(part 1 of 2)
# Autodesk Inventor assembly: Rebuild Chassis Assembly 26x28 Version with Shooter Tower
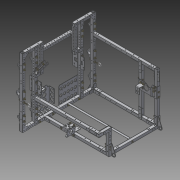
[picture p0: Inventor's stored thumbnail of the model, 180x180]
Saved by Autodesk Inventor 2014 SP1 (Build 180222100, 222)
## iProperties
Created: 2013-01-06
Part Number: Rebuild Chassis Assembly 26x28 Version with Shooter Tower
Document SubType Name: Assembly
Designer: Moses
Mass: 8941.51 g
Surface Area: 25286.9 cm^2
Volume: 3020.66 cm^3
Density: 2.96012 g/cm^3
Author: Moses
## Documents named in this file (57)
- C:\Users\Moses\Documents\Inventor\Sally Rebuild\Rebuild Sally\Rebuild Chassis Assembly 26x28 Version with Shooter Tower.iam
- C:\Users\Moses\Documents\Inventor\Sally Rebuild\Rebuild Sally\Chassis V1.500 Part3-mirror.ipt
- C:\Users\Moses\Documents\Inventor\Sally Rebuild\Rebuild Sally\Chassis V1.500 Part2.ipt
- C:\Users\Moses\Documents\Inventor\Sally Rebuild\Rebuild Sally\Chassis V1.500 Part3.ipt
- C:\Users\Moses\Documents\Inventor\Sally Rebuild\Rebuild Sally\Chassis Connector Plate V1.500.ipt
- C:\Users\Moses\Documents\Inventor\Sally Rebuild\Rebuild Sally\Chassis Corner Plate V1.500.ipt
- C:\Users\Moses\Documents\Inventor\Sally Rebuild\Rebuild Sally\Chassis Part4 (26x28).ipt
- C:\Users\Moses\Documents\Inventor\Sally Rebuild\Rebuild Sally\Chassis Part1 (26x28).ipt
- C:\Users\Moses\Documents\Inventor\Sally Rebuild\Rebuild Sally\Chassis Battery Mount Part1.ipt
- C:\Users\Moses\Documents\Inventor\Sally Rebuild\Rebuild Sally\Chassis Part9 (26x28).ipt
- C:\Users\Moses\Documents\Inventor\Sally Rebuild\Rebuild Sally\Chassis Part10 (26x28).ipt
- C:\Users\Moses\Documents\Inventor\Sally Rebuild\Rebuild Sally\Chassis Part 11 (26x28).ipt
- C:\Users\Moses\Documents\Inventor\Sally Rebuild\Rebuild Sally\Chassis Part 12 (26x28).ipt
- C:\Users\Moses\Documents\Inventor\Sally Rebuild\Rebuild Sally\Chassis Tower Bracket Part3.ipt
- C:\Users\Moses\Documents\Inventor\Sally Rebuild\Rebuild Sally\Chassis Tower Bracket Part2.ipt
- C:\Users\Moses\Documents\Inventor\Sally Rebuild\Rebuild Sally\Chassis Tower Bracket Part1.ipt
- C:\Users\Moses\Documents\Inventor\Sally Rebuild\Rebuild Sally\Rebuild Gusset 4.ipt
- C:\Users\Moses\Documents\Inventor\Sally Rebuild\Rebuild Sally\Rebuild Edge Mount 1.ipt
- C:\Users\Moses\Documents\Inventor\Sally Rebuild\Rebuild Sally\Rebuild Edge Mount 2.ipt
- C:\Users\Moses\Documents\Inventor\Sally Rebuild\Rebuild Sally\Rebuild Edge Mount 3.ipt
- C:\Users\Moses\Documents\Inventor\Sally Rebuild\Rebuild Sally\Rebuild Edge Mount 4.ipt
- C:\Users\Moses\Documents\Inventor\Sally Rebuild\Rebuild Sally\Rebuild Gusset.ipt
- C:\Users\Moses\Documents\Inventor\Sally Rebuild\Rebuild Sally\Rebuild Gusset 2.ipt
- C:\Users\Moses\Documents\Inventor\Sally Rebuild\Rebuild Sally\Gusset 3.ipt
- C:\Users\Moses\Documents\Inventor\Sally Rebuild\Rebuild Sally\Square Tube 6.ipt
- C:\Users\Moses\Documents\Inventor\Sally Rebuild\Rebuild Sally\Square Tube 3.ipt
- C:\Users\Moses\Documents\Inventor\Sally Rebuild\Rebuild Sally\Rebuild Shooter Tower Top Tube 2.ipt
- C:\Users\Moses\Documents\Inventor\Sally Rebuild\Rebuild Sally\Rebuild Gusset Connector 2.ipt
- C:\Users\Moses\Documents\Inventor\Sally Rebuild\Rebuild Sally\Rebuild Shooter Tower Top Tube 1.ipt
- C:\Users\Moses\Documents\Inventor\Sally Rebuild\Rebuild Sally\Rebuild Shooter Tower Motor Mount Tube.ipt
- C:\Users\Moses\Documents\Inventor\Sally Rebuild\Rebuild Sally\Shaft Mount V1.500 Drivetrain.ipt
- C:\Users\Moses\Documents\Inventor\Sally Rebuild\Rebuild Sally\Bearing Block V1.500 Drivetrain.ipt
- C:\Users\Moses\Documents\Inventor\Sally Rebuild\Rebuild Sally\Wheel Mount Support Plate - drive wheel.ipt
- C:\Users\Moses\Documents\Inventor\Sally Rebuild\Rebuild Sally\Wheel Mount Support Plate.ipt
- C:\Users\Moses\Documents\Inventor\Sally Rebuild\Rebuild Sally\Standard High-Strength Steel Cap Screw 0.25-20 Thread\Thread Length 0.75 - 1 in\2.000 in 91257A550\91257A550.ipt
- C:\Users\Moses\Documents\Inventor\Sally Rebuild\Rebuild Sally\Standard High-Strength Steel Cap Screw 0.25-20 Thread\90630A110.ipt
- C:\Users\Moses\Documents\Inventor\Sally Rebuild\Rebuild Sally\0.25x20 Washer.ipt
- C:\Users\Moses\Documents\Inventor\Sally Rebuild\Rebuild Sally\Standard High-Strength Steel Cap Screw 0.25-20 Thread\Thread Length 0.75 - 1 in\2.250 in 91257A551\91257A551.ipt
- C:\Users\Moses\Documents\Inventor\Sally Rebuild\Rebuild Sally\Standard High-Strength Steel Cap Screw 0.25-20 Thread\Thread Length 0.75 - 1 in\1.750 in 91257A548\91257A548.ipt
- C:\Users\Moses\Documents\Inventor\Sally Rebuild\Rebuild Sally\Rebuild Flange Bearing Mount Tower.ipt
- C:\Users\Moses\Documents\Inventor\Sally Rebuild\Rebuild Sally\Rebuild Flange Bearing Mount Tower Mirror.ipt
- C:\Users\Moses\Documents\Inventor\Sally Rebuild\Rebuild Sally\Mounting Bracket V1.500 - (toughbox-mini - sheet metal).ipt
- C:\Users\Moses\Documents\Inventor\Sally Rebuild\Rebuild Sally\Mounting Bracket V1.500 - (toughbox-mini - sheet metal - underside).ipt
- C:\Users\Moses\Documents\Inventor\Sally Rebuild\Rebuild Sally\Rebuild Mounting Board 3.ipt
- C:\Users\Moses\Documents\Inventor\Sally Rebuild\Rebuild Sally\Back Brace Mount V2.ipt
- C:\Users\Moses\Documents\Inventor\Sally Rebuild\Rebuild Sally\Circuit Breaker Mount.ipt
- C:\Users\Moses\Documents\Inventor\Sally Rebuild\Rebuild Sally\Standard High-Strength Steel Cap Screw 0.25-20 Thread\Fully Threaded\0.750 in 92620A540\92620A540.ipt
- C:\Users\Moses\Documents\Inventor\Sally Rebuild\Rebuild Sally\Rebuild Snowblower Motor Mount.ipt
- C:\Users\Moses\Documents\Inventor\Sally Rebuild\Rebuild Sally\Rebuild Encoder Mount 2.ipt
- C:\Users\Moses\Documents\Inventor\Sally Rebuild\Rebuild Sally\Standard High-Strength Steel Cap Screw 0.25-20 Thread\Fully Threaded\0.625 in 92620A539\92620A539.ipt
- C:\Users\Moses\Documents\Inventor\Sally Rebuild\Rebuild Sally\Chassis Back Electronics Protector Bar.ipt
- C:\Users\Moses\Documents\Inventor\Sally Rebuild\Rebuild Sally\Limit Switch Bracket Shooter Front Right Corner.ipt
- C:\Users\Moses\Documents\Inventor\Sally Rebuild\Rebuild Sally\Shooter Main Gear Guide Bar.ipt
- C:\Users\Moses\Documents\Inventor\Sally Rebuild\Rebuild Sally\Standard High-Strength Steel Cap Screw 0.25-20 Thread\Fully Threaded\1.000 in 92620A542\92620A542.ipt
- C:\Users\Moses\Documents\Inventor\Sally Rebuild\Rebuild Sally\0.25x20 Washer Large Diameter.ipt
- C:\Users\Moses\Documents\Inventor\Sally Rebuild\Rebuild Sally\Chassis_Channel_AndyMark (4.5 inch).ipt
- C:\Users\Moses\Documents\Inventor\Sally Rebuild\Rebuild Sally\3014T902.ipt
## Components (331 placed, 56 different names)
1. 0.25x20 Washer:101 — Insert:193, Insert:194
2. 91257A548:14 — Insert:194
3. Limit Switch Bracket Shooter Front Right Corner:1 — Mate:353, Mate:354, Mate:355, Insert:195, Insert:196
4. 0.25x20 Washer:102 — Insert:197, Insert:199
5. 0.25x20 Washer:103 — Insert:198, Insert:200
6. Shooter Main Gear Guide Bar:1 — Mate:356, Mate:357, Mate:358, Insert:201, Insert:202
7. 0.25x20 Washer:104 — Insert:199, Mate:356
8. 0.25x20 Washer:105 — Insert:200
9. 90630A110:47 — Insert:201
10. 90630A110:48 — Insert:202
11. 92620A542:1 — Insert:204
12. 92620A542:2 — Insert:203
13. 0.25x20 Washer Large Diameter:1 — Insert:205, Insert:206
14. 0.25x20 Washer Large Diameter:2 — Insert:206, Insert:207
15. 0.25x20 Washer Large Diameter:3 — Insert:207, Insert:208
16. 0.25x20 Washer Large Diameter:4 — Insert:208
17. 0.25x20 Washer Large Diameter:5 — Insert:209, Insert:210
18. 0.25x20 Washer Large Diameter:6 — Insert:210, Insert:211
19. 0.25x20 Washer Large Diameter:7 — Insert:211, Insert:212
20. 0.25x20 Washer Large Diameter:8 — Insert:212, Mate:359, Mate:360
21. Chassis_Channel_AndyMark (4.5 inch):1 — Mate:359, Mate:360, Insert:214, Angle:2, Mate:361, Insert:216
22. 0.25x20 Washer:106 — Insert:214
23. 90630A110:49
24. 0.25x20 Washer:107 — Insert:216
25. 90630A110:50
26. 3014T902:1 — Insert:217, Mate:362
27. 3014T902:2 — Insert:218, Mate:362
28. 0.25x20 Washer:108 — Insert:219, Insert:221
29. 0.25x20 Washer:109 — Insert:220, Insert:222
30. 90630A110:51 — Insert:221
31. 90630A110:52 — Insert:222
32. 0.25x20 Washer:110 — Insert:224
33. 90630A110:53
34. 0.25x20 Washer:111 — Insert:226
35. 90630A110:54
36. 0.25x20 Washer:112 — Insert:227, Insert:230
37. 0.25x20 Washer:113 — Insert:228, Insert:229
38. 91257A550:29 — Insert:229
39. 91257A550:30 — Insert:230
40. Chassis Part1 (26x28):1 — Mate:2, Flush:3, Flush:4, Flush:12, Mate:6, Flush:21, Flush:22, Mate:14, Flush:23, Flush:24, Mate:15, Flush:26, Mate:16, Flush:27, Flush:28, Flush:25, Mate:262, Mate:263, Mate:264, Mate:268, Mate:272, Mate:273, Mate:286, Mate:290, Mate:291, Mate:297, Mate:298, Mate:299, Mate:304, Mate:305, Mate:306, Mate:307, Mate:308, Mate:309, Insert:217, Insert:219, Insert:224
41. Chassis V1.500 Part2:1 — Mate:2, Flush:3, Flush:4, Mate:3, Flush:5, Flush:6, Mate:8, Mate:9, Flush:15, Flush:16, Mate:36, Mate:37, Mate:39, Mate:40, Mate:76, Mate:77, Mate:78, Mate:121, Mate:122, Mate:124, Mate:125, Mate:160, Mate:161, Mate:162, Mate:163, Flush:58, Mate:172, Mate:178, Flush:63, Mate:208, Mate:210, Mate:343, Insert:168, Insert:190, Flush:77
42. Chassis Part1 (26x28):2 — Mate:3, Flush:5, Flush:6, Flush:10, Mate:5, Flush:17, Mate:17, Flush:29, Flush:30, Mate:18, Flush:31, Flush:32, Mate:19, Flush:33, Flush:34, Mate:20, Flush:35, Flush:36, Mate:166, Mate:167, Mate:168, Flush:60, Mate:176, Flush:62, Mate:274, Mate:276, Mate:277, Mate:280, Mate:282, Mate:283, Mate:287, Mate:288, Mate:289, Mate:294, Mate:295, Mate:296, Mate:300, Mate:301, Mate:302, Mate:303, Mate:310, Mate:311, Insert:218, Insert:220, Insert:226
43. Chassis Part4 (26x28):1 — Flush:10, Mate:4, Flush:13, Mate:8, Flush:16, Mate:35, Mate:38, Mate:115, Mate:116, Mate:123, Mate:135, Flush:52, Mate:136, Mate:209, Mate:275, Mate:278, Mate:279, Mate:281, Mate:284, Mate:285, Mate:312, Mate:313, Mate:316, Mate:317, Mate:318, Mate:319, Mate:330, Mate:331, Mate:336, Mate:337, Mate:338, Mate:339
44. Chassis Part4 (26x28):2 — Flush:12, Flush:14, Mate:7, Mate:9, Flush:15, Mate:41, Mate:44, Mate:126, Mate:127, Mate:128, Mate:143, Flush:53, Mate:169, Mate:170, Mate:171, Mate:173, Flush:59, Mate:265, Mate:266, Mate:267, Mate:269, Mate:270, Mate:271, Mate:314, Mate:315, Mate:320, Mate:321, Mate:322, Mate:323, Mate:332, Mate:333, Mate:334, Mate:335, Mate:340, Mate:341, Insert:205, Angle:2, Mate:361, Insert:228
45. Chassis V1.500 Part3-mirror:1 — Mate:4, Mate:5, Flush:13, Mate:33, Mate:34, Mate:54, Flush:43, Flush:44, Mate:61, Mate:117, Mate:120
46. Chassis V1.500 Part3:1 — Mate:6, Flush:14, Mate:7, Mate:13, Mate:42, Mate:43, Mate:55, Flush:45, Flush:46, Mate:64, Mate:129, Mate:132
47. Chassis Corner Plate V1.500:1 — Flush:21, Mate:13, Flush:22
48. Chassis Corner Plate V1.500:2 — Mate:14, Flush:23, Flush:24
49. Chassis Corner Plate V1.500:3 — Mate:15, Flush:25, Flush:26
50. Chassis Corner Plate V1.500:4 — Mate:16, Flush:27, Flush:28
51. Chassis Corner Plate V1.500:5 — Mate:17, Flush:29, Flush:30
52. Chassis Corner Plate V1.500:6 — Mate:18, Flush:31, Flush:32, Mate:154, Mate:155, Mate:156, Mate:157, Mate:158, Mate:159, Mate:175, Flush:61
53. Chassis Corner Plate V1.500:7 — Mate:19, Flush:33, Flush:34
54. Chassis Corner Plate V1.500:8 — Mate:20, Flush:35, Flush:36
55. Chassis Connector Plate V1.500:5 — Mate:33, Mate:34, Mate:35
56. Chassis Connector Plate V1.500:6 — Mate:36, Mate:37, Mate:38
57. Chassis Connector Plate V1.500:7 — Mate:39, Mate:40, Mate:41
58. Chassis Connector Plate V1.500:8 — Mate:42, Mate:43, Mate:44
59. Chassis Connector Plate V1.500:9 — Mate:136, Mate:137
60. Chassis Connector Plate V1.500:10 — Mate:138, Mate:139
61. Chassis Connector Plate V1.500:11 — Mate:144, Mate:145
62. Chassis Connector Plate V1.500:12 — Mate:146, Mate:147
63. Chassis Part9 (26x28):1 — Mate:54, Flush:43, Flush:44, Mate:59, Mate:60, Mate:68, Flush:47, Mate:70, Flush:48, Mate:118, Mate:119, Mate:142, Mate:151, Flush:54
64. Chassis Part9 (26x28):2 — Mate:55, Flush:45, Flush:46, Mate:62, Mate:63, Mate:72, Mate:74, Flush:49, Flush:50, Mate:130, Mate:131, Mate:134, Flush:51, Mate:150, Mate:152, Flush:57, Mate:153, Insert:209, Insert:227
65. Chassis Connector Plate V1.500:14 — Mate:59, Mate:60, Mate:61
66. Chassis Connector Plate V1.500:16 — Mate:62, Mate:63, Mate:64
67. Chassis Connector Plate V1.500:17 — Mate:68, Flush:47, Mate:140, Mate:142
68. Chassis Connector Plate V1.500:18 — Mate:70, Flush:48, Mate:141
69. Chassis Connector Plate V1.500:19 — Mate:72, Flush:50, Mate:148, Mate:150
70. Chassis Connector Plate V1.500:20 — Mate:74, Flush:49, Mate:149
71. Chassis Connector Plate V1.500:21 — Mate:115, Mate:116, Mate:117
72. Chassis Connector Plate V1.500:22 — Mate:118, Mate:119, Mate:120
73. Chassis Connector Plate V1.500:23 — Mate:121, Mate:122, Mate:123
74. Chassis Connector Plate V1.500:24 — Mate:124, Mate:125, Mate:126
75. Chassis Connector Plate V1.500:25 — Mate:127, Mate:128, Mate:129
76. Chassis Connector Plate V1.500:26 — Mate:130, Mate:131, Mate:132
77. Chassis Part10 (26x28):1 — Mate:134, Flush:51, Flush:55, Flush:56, Mate:153
78. Chassis Part 11 (26x28):1 — Mate:135, Flush:52, Mate:137, Mate:138, Mate:139, Mate:140, Mate:141
79. Chassis Part 11 (26x28):2 — Mate:143, Mate:144, Mate:145, Mate:146, Mate:147, Flush:53, Mate:148, Mate:149
80. Chassis Part 12 (26x28):1 — Mate:151, Flush:54, Flush:55
81. Chassis Part 12 (26x28):2 — Mate:152, Flush:56, Flush:57
82. Chassis Back Electronics Protector Bar:1 — Insert:190, Flush:77, Insert:113, Insert:191
83. Rebuild Encoder Mount 2:1 — Mate:350, Mate:351, Mate:352, Insert:164, Insert:165
84. Gusset 3:1 — Mate:202, Mate:203, Mate:204, Mate:213
85. Gusset 3:2 — Mate:205, Mate:206, Mate:207, Mate:212
86. Square Tube 6:1 — Mate:211, Mate:212, Mate:213, Mate:217, Mate:218, Mate:219
87. Square Tube 3:1 — Mate:220, Mate:221, Mate:222, Mate:223, Mate:224, Mate:240, Mate:241, Mate:325, Mate:328, Mate:329
88. Rebuild Shooter Tower Top Tube 2:1 — Mate:214, Mate:215, Mate:216, Mate:225, Mate:226, Mate:235, Mate:236, Mate:237, Mate:238, Mate:239, Insert:193
89. Rebuild Gusset Connector 2:1 — Mate:217, Mate:218, Mate:219, Mate:221, Mate:222
90. Rebuild Shooter Tower Top Tube 1:1 — Mate:227, Mate:228, Mate:229, Mate:230, Mate:231, Mate:232, Mate:233, Mate:234, Mate:260, Mate:261, Mate:292, Mate:293, Insert:83, Insert:84, Mate:324, Mate:326, Mate:327, Flush:76, Mate:353, Mate:354, Mate:355
91. Rebuild Gusset:3 — Mate:232, Mate:233, Mate:234, Mate:235, Mate:236
92. Rebuild Gusset:4 — Mate:237, Mate:238, Mate:239, Mate:240, Mate:241
93. Rebuild Shooter Tower Motor Mount Tube:1 — Mate:245, Mate:246, Mate:247, Mate:248, Mate:249, Mate:250, Mate:251, Insert:77, Insert:78, Angle:1
94. Gusset 3:3 — Mate:242, Mate:243, Flush:72, Mate:246, Mate:248, Mate:249
95. Gusset 3:4 — Mate:244, Flush:73, Mate:250, Mate:251
96. Rebuild Snowblower Motor Mount:1 — Mate:260, Mate:261, Mate:292, Mate:293, Insert:79, Insert:80, Insert:81, Insert:82, Flush:76, Mate:350, Mate:351, Mate:352, Insert:162, Insert:188, Insert:189, Insert:167, Mate:357, Mate:358, Insert:203, Insert:204
97. Rebuild Flange Bearing Mount Tower:1 — Mate:324, Mate:326, Mate:327, Insert:172, Insert:173
98. Rebuild Flange Bearing Mount Tower Mirror:1 — Mate:325, Mate:328, Mate:329, Insert:99, Insert:100
99. Rebuild Gusset 4:1 — Mate:183, Mate:184, Mate:185, Mate:216, Mate:225
100. Rebuild Gusset 4:2 — Mate:180, Mate:181, Mate:182, Mate:214, Mate:215, Mate:226
101. Rebuild Gusset 4:3 — Mate:197, Flush:68, Flush:69, Mate:227, Mate:228, Mate:229, Insert:93, Insert:94
102. Rebuild Gusset 4:4 — Mate:198, Flush:70, Flush:71, Mate:230, Mate:231, Insert:155, Insert:156
103. Rebuild Gusset 4:5 — Mate:194, Mate:195, Mate:196, Mate:220, Mate:223, Mate:224, Insert:95, Insert:96
104. Rebuild Gusset:1 — Mate:188, Mate:189, Mate:190, Mate:245
105. Rebuild Gusset:2 — Mate:187, Mate:192, Mate:193
106. Rebuild Gusset 2:1 — Mate:199, Mate:200, Mate:201, Mate:211
107. Rebuild Edge Mount 4:1 — Mate:173, Flush:59, Mate:174, Mate:199, Mate:200, Mate:201, Mate:202, Mate:203, Mate:204, Mate:205, Mate:206, Mate:207
108. Rebuild Edge Mount 3:1 — Mate:175, Flush:60, Flush:61, Mate:180, Mate:181, Mate:182, Mate:188, Mate:189, Mate:190, Mate:197, Flush:68, Flush:69, Mate:242, Mate:243, Flush:72, Mate:247
109. Rebuild Edge Mount 2:1 — Mate:176, Flush:62, Mate:177, Mate:187, Mate:192, Mate:193, Mate:198, Flush:70, Flush:71, Mate:244, Flush:73
110. Rebuild Edge Mount 1:2 — Mate:178, Mate:179, Flush:63, Mate:183, Mate:184, Mate:185, Mate:194, Mate:195, Mate:196, Mate:342, Flush:75, Insert:133, Insert:135
111. Chassis Tower Bracket Part1:2 — Mate:169, Mate:170, Mate:171, Mate:174
112. Chassis Tower Bracket Part1:1 — Mate:166, Mate:167, Mate:168, Mate:177
113. Chassis Tower Bracket Part2:2 — Mate:160, Mate:161, Mate:162, Mate:179, Insert:105
114. Chassis Tower Bracket Part2:1 — Mate:163, Flush:58, Mate:172, Insert:109
115. Chassis Tower Bracket Part3:2 — Mate:154, Mate:155, Mate:156
116. Chassis Tower Bracket Part3:1 — Mate:157, Mate:158, Mate:159
117. 90630A110:46 — Insert:192
118. 0.25x20 Washer:100 — Insert:191, Insert:192
119. 0.25x20 Washer:99 — Insert:198
120. 0.25x20 Washer:98
121. 0.25x20 Washer:97
122. 0.25x20 Washer:96
123. 0.25x20 Washer:91 — Insert:197
124. 0.25x20 Washer:86 — Insert:175, Insert:176
125. 0.25x20 Washer:81 — Insert:170, Insert:171
126. 0.25x20 Washer:80 — Insert:168, Insert:169
127. 90630A110:45 — Insert:169
128. 91257A548:13 — Insert:171
129. 0.25x20 Washer:82 — Insert:97, Insert:172
130. 0.25x20 Washer:83 — Insert:98, Insert:173
131. 0.25x20 Washer:84 — Insert:174, Insert:188
132. 0.25x20 Washer:85 — Insert:174, Insert:175
133. 0.25x20 Washer:87 — Insert:176, Insert:177
134. 0.25x20 Washer:88 — Insert:177, Insert:180
135. 0.25x20 Washer:89 — Insert:180
136. 0.25x20 Washer:90
137. 0.25x20 Washer:92 — Insert:189
138. 0.25x20 Washer:94
139. 0.25x20 Washer:93
140. 0.25x20 Washer:95
141. 90630A110:43 — Insert:161
142. 0.25x20 Washer:77 — Insert:162, Insert:163
143. 92620A540:3 — Insert:163
144. 90630A110:44 — Insert:166
145. 0.25x20 Washer:78 — Insert:164, Insert:166
146. 0.25x20 Washer:79 — Insert:165, Insert:161
147. 92620A539:1 — Insert:167, Angle:1
148. 0.25x20 Washer:73 — Insert:158, Insert:195
149. 0.25x20 Washer:74 — Insert:157, Insert:196
150. 0.25x20 Washer:75 — Insert:156, Insert:160
151. 0.25x20 Washer:76 — Insert:155, Insert:159
152. 91257A548:11 — Insert:157
153. 91257A548:12 — Insert:158
154. 90630A110:41 — Insert:160
155. 90630A110:42 — Insert:159
156. 90630A110:39 — Insert:152
157. 90630A110:40 — Insert:151
158. 92620A540:2 — Insert:149
159. 92620A540:1 — Insert:150
160. 0.25x20 Washer:69 — Insert:139, Insert:151
161. 0.25x20 Washer:70 — Insert:140, Insert:152
162. 0.25x20 Washer:71 — Insert:141, Insert:149
163. 0.25x20 Washer:72 — Insert:142, Insert:150
164. 91257A548:8 — Insert:143
165. 91257A548:10 — Insert:145
166. 90630A110:36 — Insert:148
167. 90630A110:38 — Insert:146
168. 0.25x20 Washer:63 — Insert:135, Insert:146
169. 0.25x20 Washer:65 — Insert:133, Insert:148
170. 0.25x20 Washer:66 — Insert:136, Insert:143
171. 0.25x20 Washer:68 — Insert:138, Insert:145
172. 90630A110:32 — Insert:129
173. 90630A110:33 — Insert:130
174. 90630A110:34 — Insert:131
175. 90630A110:35 — Insert:132
176. 91257A550:28 — Insert:128
177. 91257A550:27 — Insert:127
178. 91257A550:26 — Insert:126
179. 91257A550:25 — Insert:125
180. 0.25x20 Washer:62 — Insert:124, Insert:131
181. 0.25x20 Washer:61 — Insert:123, Insert:132
182. 0.25x20 Washer:60 — Insert:121, Insert:129
183. 0.25x20 Washer:58 — Insert:120, Insert:128
184. 0.25x20 Washer:59 — Insert:122, Insert:130
185. 0.25x20 Washer:57 — Insert:119, Insert:127
186. 0.25x20 Washer:56 — Insert:117, Insert:125
187. 0.25x20 Washer:55 — Insert:118, Insert:126
188. 91257A550:21 — Insert:99
189. 91257A550:22 — Insert:100
190. 91257A550:23 — Insert:97
191. 91257A550:24 — Insert:98
192. 91257A548:4 — Insert:88
193. 91257A548:3 — Insert:87
194. 91257A548:2 — Insert:86
195. 91257A548:1 — Insert:85
196. 0.25x20 Washer:49 — Insert:105, Insert:108
197. 0.25x20 Washer:50 — Insert:106, Insert:107
198. 91257A548:5 — Insert:107
199. 0.25x20 Washer:51 — Insert:109, Insert:112
200. 0.25x20 Washer:52 — Insert:110, Insert:111
201. 91257A548:6 — Insert:111
202. 0.25x20 Washer:53 — Insert:113, Insert:115
203. 0.25x20 Washer:54 — Insert:114, Insert:116
204. 91257A548:7 — Insert:116
205. 90630A110:1 — Insert:57
206. 90630A110:2 — Insert:58
207. 90630A110:3 — Insert:59
208. 90630A110:4 — Insert:60
209. 90630A110:5 — Insert:62
210. 90630A110:6 — Insert:61
211. 90630A110:7 — Insert:64
212. 90630A110:8 — Insert:63
213. 90630A110:9 — Insert:66
214. 90630A110:10 — Insert:65
215. 90630A110:11 — Insert:68
216. 90630A110:12 — Insert:67
217. 90630A110:13 — Insert:69
218. 90630A110:14 — Insert:70
219. 90630A110:15 — Insert:71
220. 90630A110:16 — Insert:72
221. 90630A110:17 — Insert:73
222. 90630A110:18 — Insert:74
223. 90630A110:19 — Insert:75
224. 90630A110:20 — Insert:76
225. 90630A110:21 — Insert:90
226. 90630A110:22 — Insert:89
227. 90630A110:23 — Insert:92
228. 90630A110:24 — Insert:91
229. 90630A110:25 — Insert:102
230. 90630A110:26 — Insert:101
231. 90630A110:27 — Insert:103
232. 90630A110:28 — Insert:104
233. 90630A110:29 — Insert:108
234. 90630A110:30 — Insert:112
235. 90630A110:31 — Insert:115
236. 0.25x20 Washer:45 — Insert:93, Insert:101
237. 0.25x20 Washer:46 — Insert:94, Insert:102
238. 0.25x20 Washer:47 — Insert:96, Insert:103
239. 0.25x20 Washer:48 — Insert:95, Insert:104
240. 0.25x20 Washer:44 — Insert:84, Insert:90
241. 0.25x20 Washer:43 — Insert:83, Insert:89
242. 0.25x20 Washer:42 — Insert:82, Insert:86
243. 0.25x20 Washer:41 — Insert:81, Insert:85
244. 0.25x20 Washer:40 — Insert:80, Insert:92
245. 0.25x20 Washer:39 — Insert:79, Insert:91
246. 0.25x20 Washer:38 — Insert:77, Insert:88
247. 0.25x20 Washer:37 — Insert:78, Insert:87
248. 0.25x20 Washer:36 — Insert:48, Insert:73
249. 0.25x20 Washer:34 — Insert:56, Insert:75
250. 0.25x20 Washer:35 — Insert:47, Insert:74
251. 0.25x20 Washer:33 — Insert:55, Insert:76
252. 0.25x20 Washer:32 — Insert:50, Insert:71
253. 0.25x20 Washer:31 — Insert:49, Insert:72
254. 0.25x20 Washer:30 — Insert:52, Insert:69
255. 0.25x20 Washer:29 — Insert:51, Insert:70
256. 0.25x20 Washer:28 — Insert:54, Insert:68
257. 0.25x20 Washer:27 — Insert:53, Insert:67
258. 0.25x20 Washer:26 — Insert:44, Insert:64
259. 0.25x20 Washer:25 — Insert:43, Insert:63
260. 0.25x20 Washer:24 — Insert:45, Insert:59
261. 0.25x20 Washer:23 — Insert:46, Insert:60
262. 0.25x20 Washer:22 — Insert:41, Insert:62
263. 0.25x20 Washer:21 — Insert:42, Insert:61
264. 0.25x20 Washer:20 — Insert:40, Insert:66
265. 0.25x20 Washer:19 — Insert:39, Insert:65
266. 0.25x20 Washer:18 — Insert:38, Insert:57
267. 0.25x20 Washer:17 — Insert:37, Insert:58
268. 0.25x20 Washer:16 — Insert:36
269. 0.25x20 Washer:15 — Insert:35
270. 0.25x20 Washer:14 — Insert:34
271. 0.25x20 Washer:13 — Insert:33
272. 0.25x20 Washer:12 — Insert:32
273. 0.25x20 Washer:11 — Insert:31
274. 0.25x20 Washer:10 — Insert:30
275. 0.25x20 Washer:9 — Insert:29
276. 0.25x20 Washer:8 — Insert:28
277. 0.25x20 Washer:7 — Insert:27
278. 0.25x20 Washer:6 — Insert:26
279. 0.25x20 Washer:5 — Insert:25
280. 0.25x20 Washer:4 — Insert:24
281. 0.25x20 Washer:3 — Insert:23
282. 0.25x20 Washer:2 — Insert:22
283. 0.25x20 Washer:1 — Insert:21
284. 91257A551:3 — Insert:1
285. 91257A551:4 — Insert:2
286. 91257A551:2 — Insert:3
287. 91257A551:1 — Insert:4
288. 91257A550:5
289. 91257A550:6
290. 91257A550:7
291. 91257A550:8
292. 91257A550:9
293. 91257A550:10
294. 91257A550:11
295. 91257A550:12
296. 91257A550:13
297. 91257A550:16
298. 91257A550:15
299. 91257A550:14
300. 91257A550:17
301. 91257A550:18
302. 91257A550:19
303. 91257A550:20
304. Circuit Breaker Mount:1 — Mate:344, Mate:345, Mate:346, Insert:142, Insert:141
305. Back Brace Mount V2:1 — Mate:342, Flush:75, Mate:343, Mate:344, Mate:345, Mate:346, Insert:136, Insert:138, Insert:139, Insert:140
306. Rebuild Mounting Board 3:1 — Mate:208, Mate:209, Mate:210, Insert:114, Insert:170
307. Chassis Battery Mount Part1:1 — Mate:76, Mate:77, Mate:78, Insert:106, Insert:110
308. Mounting Bracket V1.500 - (toughbox-mini - sheet metal):1 — Mate:331, Mate:336, Mate:337, Insert:119, Insert:120
309. Mounting Bracket V1.500 - (toughbox-mini - sheet metal):2 — Mate:333, Mate:334, Mate:335, Insert:117, Insert:118
310. Mounting Bracket V1.500 - (toughbox-mini - sheet metal - underside):1 — Mate:332, Mate:340, Mate:341, Insert:121, Insert:122
311. Mounting Bracket V1.500 - (toughbox-mini - sheet metal - underside):2 — Mate:330, Mate:338, Mate:339, Insert:123, Insert:124
312. Shaft Mount V1.500 Drivetrain:1 — Mate:265, Mate:266, Mate:267, Insert:33, Insert:34
313. Shaft Mount V1.500 Drivetrain:2 — Mate:262, Mate:263, Mate:264, Insert:25, Insert:26
314. Shaft Mount V1.500 Drivetrain:3 — Mate:268, Mate:272, Mate:273, Insert:27, Insert:28
315. Shaft Mount V1.500 Drivetrain:4 — Mate:269, Mate:270, Mate:271, Insert:35, Insert:36
316. Shaft Mount V1.500 Drivetrain:5 — Mate:274, Mate:276, Mate:277, Insert:21, Insert:22
317. Shaft Mount V1.500 Drivetrain:6 — Mate:275, Mate:278, Mate:279, Insert:29, Insert:30
318. Shaft Mount V1.500 Drivetrain:7 — Mate:281, Mate:284, Mate:285, Insert:31, Insert:32
319. Shaft Mount V1.500 Drivetrain:8 — Mate:280, Mate:282, Mate:283, Insert:23, Insert:24
320. Bearing Block V1.500 Drivetrain:1 — Mate:286, Mate:290, Mate:291, Insert:3, Insert:4
321. Bearing Block V1.500 Drivetrain:2 — Mate:287, Mate:288, Mate:289, Insert:1, Insert:2
322. Wheel Mount Support Plate - drive wheel:1 — Mate:298, Mate:308, Mate:309, Insert:49, Insert:50
323. Wheel Mount Support Plate:1 — Mate:297, Mate:304, Mate:305, Insert:51, Insert:52
324. Wheel Mount Support Plate:2 — Mate:299, Mate:306, Mate:307, Insert:55, Insert:56
325. Wheel Mount Support Plate - drive wheel:2 — Mate:294, Mate:310, Mate:311, Insert:39, Insert:40
326. Wheel Mount Support Plate:3 — Mate:295, Mate:300, Mate:301, Insert:37, Insert:38
327. Wheel Mount Support Plate:4 — Mate:296, Mate:302, Mate:303, Insert:41, Insert:42
328. Wheel Mount Support Plate:5 — Mate:313, Mate:316, Mate:317, Insert:45, Insert:46
329. Wheel Mount Support Plate:6 — Mate:312, Mate:318, Mate:319, Insert:43, Insert:44
330. Wheel Mount Support Plate:7 — Mate:314, Mate:320, Mate:321, Insert:53, Insert:54
331. Wheel Mount Support Plate:8 — Mate:315, Mate:322, Mate:323, Insert:47, Insert:48
## Relationships (558: Mate 275, Insert 224, Flush 57, Angle 2)
- Mate:2: Chassis Part1 (26x28):1 ↔ Chassis V1.500 Part2:1
- Flush:3: Chassis Part1 (26x28):1 ↔ Chassis V1.500 Part2:1
- Flush:4: Chassis Part1 (26x28):1 ↔ Chassis V1.500 Part2:1
- Mate:3: Chassis V1.500 Part2:1 ↔ Chassis Part1 (26x28):2
- Flush:5: Chassis V1.500 Part2:1 ↔ Chassis Part1 (26x28):2
- Flush:6: Chassis V1.500 Part2:1 ↔ Chassis Part1 (26x28):2
- Flush:10 (-120.65 mm): Chassis Part1 (26x28):2 ↔ Chassis Part4 (26x28):1
- Flush:12 (-120.65 mm): Chassis Part1 (26x28):1 ↔ Chassis Part4 (26x28):2
- Mate:4: Chassis Part4 (26x28):1 ↔ Chassis V1.500 Part3-mirror:1
- Mate:5: Chassis Part1 (26x28):2 ↔ Chassis V1.500 Part3-mirror:1
- Flush:13: Chassis Part4 (26x28):1 ↔ Chassis V1.500 Part3-mirror:1
- Mate:6: Chassis Part1 (26x28):1 ↔ Chassis V1.500 Part3:1
- Flush:14: Chassis Part4 (26x28):2 ↔ Chassis V1.500 Part3:1
- Mate:7: Chassis Part4 (26x28):2 ↔ Chassis V1.500 Part3:1
- Mate:8: Chassis V1.500 Part2:1 ↔ Chassis Part4 (26x28):1
- Mate:9: Chassis V1.500 Part2:1 ↔ Chassis Part4 (26x28):2
- Flush:15: Chassis V1.500 Part2:1 ↔ Chassis Part4 (26x28):2
- Flush:16: Chassis V1.500 Part2:1 ↔ Chassis Part4 (26x28):1
- Flush:17 (330.2 mm): Chassis Part1 (26x28):2
- Flush:21: Chassis Part1 (26x28):1 ↔ Chassis Corner Plate V1.500:1
- Mate:13: Chassis V1.500 Part3:1 ↔ Chassis Corner Plate V1.500:1
- Flush:22: Chassis Part1 (26x28):1 ↔ Chassis Corner Plate V1.500:1
- Mate:14: Chassis Part1 (26x28):1 ↔ Chassis Corner Plate V1.500:2
- Flush:23: Chassis Part1 (26x28):1 ↔ Chassis Corner Plate V1.500:2
- Flush:24: Chassis Part1 (26x28):1 ↔ Chassis Corner Plate V1.500:2
- Mate:15: Chassis Part1 (26x28):1 ↔ Chassis Corner Plate V1.500:3
- Flush:25: Chassis Part1 (26x28):1 ↔ Chassis Corner Plate V1.500:3
- Flush:26: Chassis Part1 (26x28):1 ↔ Chassis Corner Plate V1.500:3
- Mate:16: Chassis Part1 (26x28):1 ↔ Chassis Corner Plate V1.500:4
- Flush:27: Chassis Part1 (26x28):1 ↔ Chassis Corner Plate V1.500:4
- Flush:28: Chassis Part1 (26x28):1 ↔ Chassis Corner Plate V1.500:4
- Mate:17: Chassis Part1 (26x28):2 ↔ Chassis Corner Plate V1.500:5
- Flush:29: Chassis Part1 (26x28):2 ↔ Chassis Corner Plate V1.500:5
- Flush:30: Chassis Part1 (26x28):2 ↔ Chassis Corner Plate V1.500:5
- Mate:18: Chassis Part1 (26x28):2 ↔ Chassis Corner Plate V1.500:6
- Flush:31: Chassis Part1 (26x28):2 ↔ Chassis Corner Plate V1.500:6
- Flush:32: Chassis Part1 (26x28):2 ↔ Chassis Corner Plate V1.500:6
- Mate:19: Chassis Part1 (26x28):2 ↔ Chassis Corner Plate V1.500:7
- Flush:33: Chassis Part1 (26x28):2 ↔ Chassis Corner Plate V1.500:7
- Flush:34: Chassis Part1 (26x28):2 ↔ Chassis Corner Plate V1.500:7
- Mate:20: Chassis Part1 (26x28):2 ↔ Chassis Corner Plate V1.500:8
- Flush:35: Chassis Part1 (26x28):2 ↔ Chassis Corner Plate V1.500:8
- Flush:36: Chassis Part1 (26x28):2 ↔ Chassis Corner Plate V1.500:8
- Mate:33: Chassis V1.500 Part3-mirror:1 ↔ Chassis Connector Plate V1.500:5
- Mate:34: Chassis V1.500 Part3-mirror:1 ↔ Chassis Connector Plate V1.500:5
- Mate:35: Chassis Part4 (26x28):1 ↔ Chassis Connector Plate V1.500:5
- Mate:36: Chassis V1.500 Part2:1 ↔ Chassis Connector Plate V1.500:6
- Mate:37: Chassis V1.500 Part2:1 ↔ Chassis Connector Plate V1.500:6
- Mate:38: Chassis Part4 (26x28):1 ↔ Chassis Connector Plate V1.500:6
- Mate:39: Chassis V1.500 Part2:1 ↔ Chassis Connector Plate V1.500:7
- Mate:40: Chassis V1.500 Part2:1 ↔ Chassis Connector Plate V1.500:7
- Mate:41: Chassis Part4 (26x28):2 ↔ Chassis Connector Plate V1.500:7
- Mate:42: Chassis V1.500 Part3:1 ↔ Chassis Connector Plate V1.500:8
- Mate:43: Chassis V1.500 Part3:1 ↔ Chassis Connector Plate V1.500:8
- Mate:44: Chassis Part4 (26x28):2 ↔ Chassis Connector Plate V1.500:8
- Mate:54: Chassis V1.500 Part3-mirror:1 ↔ Chassis Part9 (26x28):1
- Flush:43: Chassis V1.500 Part3-mirror:1 ↔ Chassis Part9 (26x28):1
- Flush:44: Chassis V1.500 Part3-mirror:1 ↔ Chassis Part9 (26x28):1
- Mate:55: Chassis V1.500 Part3:1 ↔ Chassis Part9 (26x28):2
- Flush:45: Chassis V1.500 Part3:1 ↔ Chassis Part9 (26x28):2
- Flush:46: Chassis V1.500 Part3:1 ↔ Chassis Part9 (26x28):2
- Mate:59: Chassis Part9 (26x28):1 ↔ Chassis Connector Plate V1.500:14
- Mate:60: Chassis Part9 (26x28):1 ↔ Chassis Connector Plate V1.500:14
- Mate:61: Chassis V1.500 Part3-mirror:1 ↔ Chassis Connector Plate V1.500:14
- Mate:62: Chassis Part9 (26x28):2 ↔ Chassis Connector Plate V1.500:16
- Mate:63: Chassis Part9 (26x28):2 ↔ Chassis Connector Plate V1.500:16
- Mate:64: Chassis V1.500 Part3:1 ↔ Chassis Connector Plate V1.500:16
- Mate:68: Chassis Part9 (26x28):1 ↔ Chassis Connector Plate V1.500:17
- Flush:47: Chassis Part9 (26x28):1 ↔ Chassis Connector Plate V1.500:17
- Mate:70: Chassis Part9 (26x28):1 ↔ Chassis Connector Plate V1.500:18
- Flush:48: Chassis Part9 (26x28):1 ↔ Chassis Connector Plate V1.500:18
- Mate:72: Chassis Part9 (26x28):2 ↔ Chassis Connector Plate V1.500:19
- Mate:74: Chassis Part9 (26x28):2 ↔ Chassis Connector Plate V1.500:20
- Flush:49: Chassis Part9 (26x28):2 ↔ Chassis Connector Plate V1.500:20
- Flush:50: Chassis Part9 (26x28):2 ↔ Chassis Connector Plate V1.500:19
- Mate:76: Chassis V1.500 Part2:1 ↔ Chassis Battery Mount Part1:1
- Mate:77: Chassis V1.500 Part2:1 ↔ Chassis Battery Mount Part1:1
- Mate:78: Chassis V1.500 Part2:1 ↔ Chassis Battery Mount Part1:1
- Mate:115: Chassis Part4 (26x28):1 ↔ Chassis Connector Plate V1.500:21
- Mate:116: Chassis Part4 (26x28):1 ↔ Chassis Connector Plate V1.500:21
- Mate:117: Chassis V1.500 Part3-mirror:1 ↔ Chassis Connector Plate V1.500:21
- Mate:118: Chassis Part9 (26x28):1 ↔ Chassis Connector Plate V1.500:22
- Mate:119: Chassis Part9 (26x28):1 ↔ Chassis Connector Plate V1.500:22
- Mate:120: Chassis V1.500 Part3-mirror:1 ↔ Chassis Connector Plate V1.500:22
- Mate:121: Chassis V1.500 Part2:1 ↔ Chassis Connector Plate V1.500:23
- Mate:122: Chassis V1.500 Part2:1 ↔ Chassis Connector Plate V1.500:23
- Mate:123: Chassis Part4 (26x28):1 ↔ Chassis Connector Plate V1.500:23
- Mate:124: Chassis V1.500 Part2:1 ↔ Chassis Connector Plate V1.500:24
- Mate:125: Chassis V1.500 Part2:1 ↔ Chassis Connector Plate V1.500:24
- Mate:126: Chassis Part4 (26x28):2 ↔ Chassis Connector Plate V1.500:24
- Mate:127: Chassis Part4 (26x28):2 ↔ Chassis Connector Plate V1.500:25
- Mate:128: Chassis Part4 (26x28):2 ↔ Chassis Connector Plate V1.500:25
- Mate:129: Chassis V1.500 Part3:1 ↔ Chassis Connector Plate V1.500:25
- Mate:130: Chassis Part9 (26x28):2 ↔ Chassis Connector Plate V1.500:26
- Mate:131: Chassis Part9 (26x28):2 ↔ Chassis Connector Plate V1.500:26
- Mate:132: Chassis V1.500 Part3:1 ↔ Chassis Connector Plate V1.500:26
- Mate:134 (19.05 mm): Chassis Part9 (26x28):2 ↔ Chassis Part10 (26x28):1
- Flush:51: Chassis Part9 (26x28):2 ↔ Chassis Part10 (26x28):1
- Mate:135: Chassis Part4 (26x28):1 ↔ Chassis Part 11 (26x28):1
- Flush:52: Chassis Part4 (26x28):1 ↔ Chassis Part 11 (26x28):1
- Mate:136: Chassis Part4 (26x28):1 ↔ Chassis Connector Plate V1.500:9
- Mate:137: Chassis Connector Plate V1.500:9 ↔ Chassis Part 11 (26x28):1
- Mate:138: Chassis Connector Plate V1.500:10 ↔ Chassis Part 11 (26x28):1
- Mate:139: Chassis Connector Plate V1.500:10 ↔ Chassis Part 11 (26x28):1
- Mate:140: Chassis Connector Plate V1.500:17 ↔ Chassis Part 11 (26x28):1
- Mate:141: Chassis Connector Plate V1.500:18 ↔ Chassis Part 11 (26x28):1
- Mate:142: Chassis Part9 (26x28):1 ↔ Chassis Connector Plate V1.500:17
- Mate:143: Chassis Part4 (26x28):2 ↔ Chassis Part 11 (26x28):2
- Mate:144: Chassis Connector Plate V1.500:11 ↔ Chassis Part 11 (26x28):2
- Mate:145: Chassis Connector Plate V1.500:11 ↔ Chassis Part 11 (26x28):2
- Mate:146: Chassis Connector Plate V1.500:12 ↔ Chassis Part 11 (26x28):2
- Mate:147: Chassis Connector Plate V1.500:12 ↔ Chassis Part 11 (26x28):2
- Flush:53: Chassis Part4 (26x28):2 ↔ Chassis Part 11 (26x28):2
- Mate:148: Chassis Connector Plate V1.500:19 ↔ Chassis Part 11 (26x28):2
- Mate:149: Chassis Connector Plate V1.500:20 ↔ Chassis Part 11 (26x28):2
- Mate:150: Chassis Part9 (26x28):2 ↔ Chassis Connector Plate V1.500:19
- Mate:151: Chassis Part9 (26x28):1 ↔ Chassis Part 12 (26x28):1
- Flush:54: Chassis Part9 (26x28):1 ↔ Chassis Part 12 (26x28):1
- Flush:55: Chassis Part10 (26x28):1 ↔ Chassis Part 12 (26x28):1
- Mate:152: Chassis Part9 (26x28):2 ↔ Chassis Part 12 (26x28):2
- Flush:56: Chassis Part10 (26x28):1 ↔ Chassis Part 12 (26x28):2
- Flush:57: Chassis Part9 (26x28):2 ↔ Chassis Part 12 (26x28):2
- Mate:153: Chassis Part9 (26x28):2 ↔ Chassis Part10 (26x28):1
- Mate:154: Chassis Corner Plate V1.500:6 ↔ Chassis Tower Bracket Part3:2
- Mate:155: Chassis Corner Plate V1.500:6 ↔ Chassis Tower Bracket Part3:2
- Mate:156: Chassis Corner Plate V1.500:6 ↔ Chassis Tower Bracket Part3:2
- Mate:157: Chassis Corner Plate V1.500:6 ↔ Chassis Tower Bracket Part3:1
- Mate:158: Chassis Corner Plate V1.500:6 ↔ Chassis Tower Bracket Part3:1
- Mate:159: Chassis Corner Plate V1.500:6 ↔ Chassis Tower Bracket Part3:1
- Mate:160: Chassis V1.500 Part2:1 ↔ Chassis Tower Bracket Part2:2
- Mate:161: Chassis V1.500 Part2:1 ↔ Chassis Tower Bracket Part2:2
- Mate:162: Chassis V1.500 Part2:1 ↔ Chassis Tower Bracket Part2:2
- Mate:163: Chassis V1.500 Part2:1 ↔ Chassis Tower Bracket Part2:1
- Mate:166: Chassis Part1 (26x28):2 ↔ Chassis Tower Bracket Part1:1
- Mate:167: Chassis Part1 (26x28):2 ↔ Chassis Tower Bracket Part1:1
- Mate:168: Chassis Part1 (26x28):2 ↔ Chassis Tower Bracket Part1:1
- Mate:169: Chassis Part4 (26x28):2 ↔ Chassis Tower Bracket Part1:2
- Mate:170: Chassis Part4 (26x28):2 ↔ Chassis Tower Bracket Part1:2
- Mate:171: Chassis Part4 (26x28):2 ↔ Chassis Tower Bracket Part1:2
- Flush:58: Chassis V1.500 Part2:1 ↔ Chassis Tower Bracket Part2:1
- Mate:172: Chassis V1.500 Part2:1 ↔ Chassis Tower Bracket Part2:1
- Mate:173: Chassis Part4 (26x28):2 ↔ Rebuild Edge Mount 4:1
- Flush:59: Chassis Part4 (26x28):2 ↔ Rebuild Edge Mount 4:1
- Mate:174: Rebuild Edge Mount 4:1 ↔ Chassis Tower Bracket Part1:2
- Mate:175: Chassis Corner Plate V1.500:6 ↔ Rebuild Edge Mount 3:1
- Flush:60: Chassis Part1 (26x28):2 ↔ Rebuild Edge Mount 3:1
- Flush:61: Chassis Corner Plate V1.500:6 ↔ Rebuild Edge Mount 3:1
- Mate:176: Chassis Part1 (26x28):2 ↔ Rebuild Edge Mount 2:1
- Flush:62: Chassis Part1 (26x28):2 ↔ Rebuild Edge Mount 2:1
- Mate:177: Rebuild Edge Mount 2:1 ↔ Chassis Tower Bracket Part1:1
- Mate:178: Chassis V1.500 Part2:1 ↔ Rebuild Edge Mount 1:2
- Mate:179: Rebuild Edge Mount 1:2 ↔ Chassis Tower Bracket Part2:2
- Flush:63: Chassis V1.500 Part2:1 ↔ Rebuild Edge Mount 1:2
- Mate:180: Rebuild Gusset 4:2 ↔ Rebuild Edge Mount 3:1
- Mate:181: Rebuild Gusset 4:2 ↔ Rebuild Edge Mount 3:1
- Mate:182: Rebuild Gusset 4:2 ↔ Rebuild Edge Mount 3:1
- Mate:183: Rebuild Gusset 4:1 ↔ Rebuild Edge Mount 1:2
- Mate:184: Rebuild Gusset 4:1 ↔ Rebuild Edge Mount 1:2
- Mate:185: Rebuild Gusset 4:1 ↔ Rebuild Edge Mount 1:2
- Mate:187: Rebuild Gusset:2 ↔ Rebuild Edge Mount 2:1
- Mate:188: Rebuild Gusset:1 ↔ Rebuild Edge Mount 3:1
- Mate:189: Rebuild Gusset:1 ↔ Rebuild Edge Mount 3:1
- Mate:190: Rebuild Gusset:1 ↔ Rebuild Edge Mount 3:1
- Mate:192: Rebuild Gusset:2 ↔ Rebuild Edge Mount 2:1
- Mate:193: Rebuild Gusset:2 ↔ Rebuild Edge Mount 2:1
- Mate:194: Rebuild Gusset 4:5 ↔ Rebuild Edge Mount 1:2
- Mate:195: Rebuild Gusset 4:5 ↔ Rebuild Edge Mount 1:2
- Mate:196: Rebuild Gusset 4:5 ↔ Rebuild Edge Mount 1:2
- Mate:197: Rebuild Gusset 4:3 ↔ Rebuild Edge Mount 3:1
- Flush:68: Rebuild Gusset 4:3 ↔ Rebuild Edge Mount 3:1
- Flush:69: Rebuild Gusset 4:3 ↔ Rebuild Edge Mount 3:1
- Mate:198: Rebuild Gusset 4:4 ↔ Rebuild Edge Mount 2:1
- Flush:70: Rebuild Gusset 4:4 ↔ Rebuild Edge Mount 2:1
- Flush:71: Rebuild Gusset 4:4 ↔ Rebuild Edge Mount 2:1
- Mate:199: Rebuild Gusset 2:1 ↔ Rebuild Edge Mount 4:1
- Mate:200: Rebuild Gusset 2:1 ↔ Rebuild Edge Mount 4:1
- Mate:201: Rebuild Gusset 2:1 ↔ Rebuild Edge Mount 4:1
- Mate:202: Gusset 3:1 ↔ Rebuild Edge Mount 4:1
- Mate:203: Gusset 3:1 ↔ Rebuild Edge Mount 4:1
- Mate:204: Gusset 3:1 ↔ Rebuild Edge Mount 4:1
- Mate:205: Gusset 3:2 ↔ Rebuild Edge Mount 4:1
- Mate:206: Gusset 3:2 ↔ Rebuild Edge Mount 4:1
- Mate:207: Gusset 3:2 ↔ Rebuild Edge Mount 4:1
- Mate:208: Chassis V1.500 Part2:1 ↔ Rebuild Mounting Board 3:1
- Mate:209: Chassis Part4 (26x28):1 ↔ Rebuild Mounting Board 3:1
- Mate:210: Chassis V1.500 Part2:1 ↔ Rebuild Mounting Board 3:1
- Mate:211: Square Tube 6:1 ↔ Rebuild Gusset 2:1
- Mate:212: Gusset 3:2 ↔ Square Tube 6:1
- Mate:213: Gusset 3:1 ↔ Square Tube 6:1
- Mate:214: Rebuild Shooter Tower Top Tube 2:1 ↔ Rebuild Gusset 4:2
- Mate:215: Rebuild Shooter Tower Top Tube 2:1 ↔ Rebuild Gusset 4:2
- Mate:216: Rebuild Shooter Tower Top Tube 2:1 ↔ Rebuild Gusset 4:1
- Mate:217: Square Tube 6:1 ↔ Rebuild Gusset Connector 2:1
- Mate:218: Square Tube 6:1 ↔ Rebuild Gusset Connector 2:1
- Mate:219: Square Tube 6:1 ↔ Rebuild Gusset Connector 2:1
- Mate:220: Square Tube 3:1 ↔ Rebuild Gusset 4:5
- Mate:221: Square Tube 3:1 ↔ Rebuild Gusset Connector 2:1
- Mate:222: Square Tube 3:1 ↔ Rebuild Gusset Connector 2:1
- Mate:223: Square Tube 3:1 ↔ Rebuild Gusset 4:5
- Mate:224: Square Tube 3:1 ↔ Rebuild Gusset 4:5
- Mate:225: Rebuild Shooter Tower Top Tube 2:1 ↔ Rebuild Gusset 4:1
- Mate:226: Rebuild Shooter Tower Top Tube 2:1 ↔ Rebuild Gusset 4:2
- Mate:227: Rebuild Shooter Tower Top Tube 1:1 ↔ Rebuild Gusset 4:3
- Mate:228: Rebuild Shooter Tower Top Tube 1:1 ↔ Rebuild Gusset 4:3
- Mate:229: Rebuild Shooter Tower Top Tube 1:1 ↔ Rebuild Gusset 4:3
- Mate:230: Rebuild Shooter Tower Top Tube 1:1 ↔ Rebuild Gusset 4:4
- Mate:231: Rebuild Shooter Tower Top Tube 1:1 ↔ Rebuild Gusset 4:4
- Mate:232: Rebuild Shooter Tower Top Tube 1:1 ↔ Rebuild Gusset:3
- Mate:233: Rebuild Shooter Tower Top Tube 1:1 ↔ Rebuild Gusset:3
- Mate:234: Rebuild Shooter Tower Top Tube 1:1 ↔ Rebuild Gusset:3
- Mate:235: Rebuild Shooter Tower Top Tube 2:1 ↔ Rebuild Gusset:3
- Mate:236: Rebuild Shooter Tower Top Tube 2:1 ↔ Rebuild Gusset:3
- Mate:237: Rebuild Shooter Tower Top Tube 2:1 ↔ Rebuild Gusset:4
- Mate:238: Rebuild Shooter Tower Top Tube 2:1 ↔ Rebuild Gusset:4
- Mate:239: Rebuild Shooter Tower Top Tube 2:1 ↔ Rebuild Gusset:4
- Mate:240: Square Tube 3:1 ↔ Rebuild Gusset:4
- Mate:241: Square Tube 3:1 ↔ Rebuild Gusset:4
- Mate:242: Gusset 3:3 ↔ Rebuild Edge Mount 3:1
- Mate:243: Gusset 3:3 ↔ Rebuild Edge Mount 3:1
- Flush:72: Gusset 3:3 ↔ Rebuild Edge Mount 3:1
- Mate:244: Gusset 3:4 ↔ Rebuild Edge Mount 2:1
- Flush:73: Gusset 3:4 ↔ Rebuild Edge Mount 2:1
- Mate:245: Rebuild Shooter Tower Motor Mount Tube:1 ↔ Rebuild Gusset:1
- Mate:246: Rebuild Shooter Tower Motor Mount Tube:1 ↔ Gusset 3:3
- Mate:247: Rebuild Shooter Tower Motor Mount Tube:1 ↔ Rebuild Edge Mount 3:1
- Mate:248: Rebuild Shooter Tower Motor Mount Tube:1 ↔ Gusset 3:3
- Mate:249: Rebuild Shooter Tower Motor Mount Tube:1 ↔ Gusset 3:3
- Mate:250: Rebuild Shooter Tower Motor Mount Tube:1 ↔ Gusset 3:4
- Mate:251: Rebuild Shooter Tower Motor Mount Tube:1 ↔ Gusset 3:4
- Mate:260: Rebuild Shooter Tower Top Tube 1:1 ↔ Rebuild Snowblower Motor Mount:1
- Mate:261: Rebuild Shooter Tower Top Tube 1:1 ↔ Rebuild Snowblower Motor Mount:1
- Mate:262: Chassis Part1 (26x28):1 ↔ Shaft Mount V1.500 Drivetrain:2
- Mate:263: Chassis Part1 (26x28):1 ↔ Shaft Mount V1.500 Drivetrain:2
- Mate:264: Chassis Part1 (26x28):1 ↔ Shaft Mount V1.500 Drivetrain:2
- Mate:265: Chassis Part4 (26x28):2 ↔ Shaft Mount V1.500 Drivetrain:1
- Mate:266: Chassis Part4 (26x28):2 ↔ Shaft Mount V1.500 Drivetrain:1
- Mate:267: Chassis Part4 (26x28):2 ↔ Shaft Mount V1.500 Drivetrain:1
- Mate:268: Chassis Part1 (26x28):1 ↔ Shaft Mount V1.500 Drivetrain:3
- Mate:269: Chassis Part4 (26x28):2 ↔ Shaft Mount V1.500 Drivetrain:4
- Mate:270: Chassis Part4 (26x28):2 ↔ Shaft Mount V1.500 Drivetrain:4
- Mate:271: Chassis Part4 (26x28):2 ↔ Shaft Mount V1.500 Drivetrain:4
- Mate:272: Chassis Part1 (26x28):1 ↔ Shaft Mount V1.500 Drivetrain:3
- Mate:273: Chassis Part1 (26x28):1 ↔ Shaft Mount V1.500 Drivetrain:3
- Mate:274: Chassis Part1 (26x28):2 ↔ Shaft Mount V1.500 Drivetrain:5
- Mate:275: Chassis Part4 (26x28):1 ↔ Shaft Mount V1.500 Drivetrain:6
- Mate:276: Chassis Part1 (26x28):2 ↔ Shaft Mount V1.500 Drivetrain:5
- Mate:277: Chassis Part1 (26x28):2 ↔ Shaft Mount V1.500 Drivetrain:5
- Mate:278: Chassis Part4 (26x28):1 ↔ Shaft Mount V1.500 Drivetrain:6
- Mate:279: Chassis Part4 (26x28):1 ↔ Shaft Mount V1.500 Drivetrain:6
- Mate:280: Chassis Part1 (26x28):2 ↔ Shaft Mount V1.500 Drivetrain:8
- Mate:281: Chassis Part4 (26x28):1 ↔ Shaft Mount V1.500 Drivetrain:7
- Mate:282: Chassis Part1 (26x28):2 ↔ Shaft Mount V1.500 Drivetrain:8
- Mate:283: Chassis Part1 (26x28):2 ↔ Shaft Mount V1.500 Drivetrain:8
- Mate:284: Chassis Part4 (26x28):1 ↔ Shaft Mount V1.500 Drivetrain:7
- Mate:285: Chassis Part4 (26x28):1 ↔ Shaft Mount V1.500 Drivetrain:7
- Mate:286: Chassis Part1 (26x28):1 ↔ Bearing Block V1.500 Drivetrain:1
- Mate:287: Chassis Part1 (26x28):2 ↔ Bearing Block V1.500 Drivetrain:2
- Mate:288: Chassis Part1 (26x28):2 ↔ Bearing Block V1.500 Drivetrain:2
- Mate:289: Chassis Part1 (26x28):2 ↔ Bearing Block V1.500 Drivetrain:2
- Mate:290: Chassis Part1 (26x28):1 ↔ Bearing Block V1.500 Drivetrain:1
- Mate:291: Chassis Part1 (26x28):1 ↔ Bearing Block V1.500 Drivetrain:1
- Mate:292: Rebuild Shooter Tower Top Tube 1:1 ↔ Rebuild Snowblower Motor Mount:1
- Mate:293: Rebuild Shooter Tower Top Tube 1:1 ↔ Rebuild Snowblower Motor Mount:1
- Mate:294: Chassis Part1 (26x28):2 ↔ Wheel Mount Support Plate - drive wheel:2
- Mate:295: Chassis Part1 (26x28):2 ↔ Wheel Mount Support Plate:3
- Mate:296: Chassis Part1 (26x28):2 ↔ Wheel Mount Support Plate:4
- Mate:297: Chassis Part1 (26x28):1 ↔ Wheel Mount Support Plate:1
- Mate:298: Chassis Part1 (26x28):1 ↔ Wheel Mount Support Plate - drive wheel:1
- Mate:299: Chassis Part1 (26x28):1 ↔ Wheel Mount Support Plate:2
- Mate:300: Chassis Part1 (26x28):2 ↔ Wheel Mount Support Plate:3
- Mate:301: Chassis Part1 (26x28):2 ↔ Wheel Mount Support Plate:3
- Mate:302: Chassis Part1 (26x28):2 ↔ Wheel Mount Support Plate:4
- Mate:303: Chassis Part1 (26x28):2 ↔ Wheel Mount Support Plate:4
- Mate:304: Chassis Part1 (26x28):1 ↔ Wheel Mount Support Plate:1
- Mate:305: Chassis Part1 (26x28):1 ↔ Wheel Mount Support Plate:1
- Mate:306: Chassis Part1 (26x28):1 ↔ Wheel Mount Support Plate:2
- Mate:307: Chassis Part1 (26x28):1 ↔ Wheel Mount Support Plate:2
- Mate:308: Chassis Part1 (26x28):1 ↔ Wheel Mount Support Plate - drive wheel:1
- Mate:309: Chassis Part1 (26x28):1 ↔ Wheel Mount Support Plate - drive wheel:1
- Mate:310: Chassis Part1 (26x28):2 ↔ Wheel Mount Support Plate - drive wheel:2
- Mate:311: Chassis Part1 (26x28):2 ↔ Wheel Mount Support Plate - drive wheel:2
- Insert:1: 91257A551:3 ↔ Bearing Block V1.500 Drivetrain:2
- Insert:2: 91257A551:4 ↔ Bearing Block V1.500 Drivetrain:2
- Insert:3: 91257A551:2 ↔ Bearing Block V1.500 Drivetrain:1
- Insert:4: 91257A551:1 ↔ Bearing Block V1.500 Drivetrain:1
- [Insert]: 0.25x20 Washer:2 ↔ 91257A550:5
- [Insert]: 0.25x20 Washer:1 ↔ 91257A550:6
- [Insert]: 0.25x20 Washer:4 ↔ 91257A550:7
- [Insert]: 0.25x20 Washer:3 ↔ 91257A550:8
- [Insert]: 0.25x20 Washer:6 ↔ 91257A550:9
- [Insert]: 0.25x20 Washer:5 ↔ 91257A550:10
- [Insert]: 0.25x20 Washer:7 ↔ 91257A550:11
- [Insert]: 0.25x20 Washer:8 ↔ 91257A550:12
- [Insert]: 0.25x20 Washer:10 ↔ 91257A550:14
- [Insert]: 0.25x20 Washer:9 ↔ 91257A550:13
- [Insert]: 0.25x20 Washer:11 ↔ 91257A550:15
- [Insert]: 0.25x20 Washer:12 ↔ 91257A550:16
- [Insert]: 0.25x20 Washer:13 ↔ 91257A550:18
- [Insert]: 0.25x20 Washer:14 ↔ 91257A550:17
- [Insert]: 0.25x20 Washer:15 ↔ 91257A550:19
- [Insert]: 0.25x20 Washer:16 ↔ 91257A550:20
- Insert:21: 0.25x20 Washer:1 ↔ Shaft Mount V1.500 Drivetrain:5
- Insert:22: 0.25x20 Washer:2 ↔ Shaft Mount V1.500 Drivetrain:5
- Insert:23: 0.25x20 Washer:3 ↔ Shaft Mount V1.500 Drivetrain:8
- Insert:24: 0.25x20 Washer:4 ↔ Shaft Mount V1.500 Drivetrain:8
- Insert:25: 0.25x20 Washer:5 ↔ Shaft Mount V1.500 Drivetrain:2
- Insert:26: 0.25x20 Washer:6 ↔ Shaft Mount V1.500 Drivetrain:2
- Insert:27: 0.25x20 Washer:7 ↔ Shaft Mount V1.500 Drivetrain:3
- Insert:28: 0.25x20 Washer:8 ↔ Shaft Mount V1.500 Drivetrain:3
- Insert:29: 0.25x20 Washer:9 ↔ Shaft Mount V1.500 Drivetrain:6
- Insert:30: 0.25x20 Washer:10 ↔ Shaft Mount V1.500 Drivetrain:6
- Insert:31: 0.25x20 Washer:11 ↔ Shaft Mount V1.500 Drivetrain:7
- Insert:32: 0.25x20 Washer:12 ↔ Shaft Mount V1.500 Drivetrain:7
- Insert:33: 0.25x20 Washer:13 ↔ Shaft Mount V1.500 Drivetrain:1
- Insert:34: 0.25x20 Washer:14 ↔ Shaft Mount V1.500 Drivetrain:1
- Insert:35: 0.25x20 Washer:15 ↔ Shaft Mount V1.500 Drivetrain:4
- Insert:36: 0.25x20 Washer:16 ↔ Shaft Mount V1.500 Drivetrain:4
- Insert:37: 0.25x20 Washer:17 ↔ Wheel Mount Support Plate:3
- Insert:38: 0.25x20 Washer:18 ↔ Wheel Mount Support Plate:3
- Insert:39: 0.25x20 Washer:19 ↔ Wheel Mount Support Plate - drive wheel:2
- Insert:40: 0.25x20 Washer:20 ↔ Wheel Mount Support Plate - drive wheel:2
- Insert:41: 0.25x20 Washer:22 ↔ Wheel Mount Support Plate:4
- Insert:42: 0.25x20 Washer:21 ↔ Wheel Mount Support Plate:4
- Mate:312: Chassis Part4 (26x28):1 ↔ Wheel Mount Support Plate:6
- Mate:313: Chassis Part4 (26x28):1 ↔ Wheel Mount Support Plate:5
- Mate:314: Chassis Part4 (26x28):2 ↔ Wheel Mount Support Plate:7
- Mate:315: Chassis Part4 (26x28):2 ↔ Wheel Mount Support Plate:8
- Mate:316: Chassis Part4 (26x28):1 ↔ Wheel Mount Support Plate:5
- Mate:317: Chassis Part4 (26x28):1 ↔ Wheel Mount Support Plate:5
- Mate:318: Chassis Part4 (26x28):1 ↔ Wheel Mount Support Plate:6
- Mate:319: Chassis Part4 (26x28):1 ↔ Wheel Mount Support Plate:6
- Mate:320: Chassis Part4 (26x28):2 ↔ Wheel Mount Support Plate:7
- Mate:321: Chassis Part4 (26x28):2 ↔ Wheel Mount Support Plate:7
- Mate:322: Chassis Part4 (26x28):2 ↔ Wheel Mount Support Plate:8
- Mate:323: Chassis Part4 (26x28):2 ↔ Wheel Mount Support Plate:8
- Insert:43: 0.25x20 Washer:25 ↔ Wheel Mount Support Plate:6
- Insert:44: 0.25x20 Washer:26 ↔ Wheel Mount Support Plate:6
- Insert:45: 0.25x20 Washer:24 ↔ Wheel Mount Support Plate:5
- Insert:46: 0.25x20 Washer:23 ↔ Wheel Mount Support Plate:5
- Insert:47: 0.25x20 Washer:35 ↔ Wheel Mount Support Plate:8
- Insert:48: 0.25x20 Washer:36 ↔ Wheel Mount Support Plate:8
- Insert:49: 0.25x20 Washer:31 ↔ Wheel Mount Support Plate - drive wheel:1
- Insert:50: 0.25x20 Washer:32 ↔ Wheel Mount Support Plate - drive wheel:1
- Insert:51: 0.25x20 Washer:29 ↔ Wheel Mount Support Plate:1
- Insert:52: 0.25x20 Washer:30 ↔ Wheel Mount Support Plate:1
- Insert:53: 0.25x20 Washer:27 ↔ Wheel Mount Support Plate:7
- Insert:54: 0.25x20 Washer:28 ↔ Wheel Mount Support Plate:7
- Insert:55: 0.25x20 Washer:33 ↔ Wheel Mount Support Plate:2
- Insert:56: 0.25x20 Washer:34 ↔ Wheel Mount Support Plate:2
- Insert:57: 90630A110:1 ↔ 0.25x20 Washer:18
- Insert:58: 90630A110:2 ↔ 0.25x20 Washer:17
- Insert:59: 90630A110:3 ↔ 0.25x20 Washer:24
- Insert:60: 90630A110:4 ↔ 0.25x20 Washer:23
- Insert:61: 90630A110:6 ↔ 0.25x20 Washer:21
- Insert:62: 90630A110:5 ↔ 0.25x20 Washer:22
- Insert:63: 90630A110:8 ↔ 0.25x20 Washer:25
- Insert:64: 90630A110:7 ↔ 0.25x20 Washer:26
- Insert:65: 90630A110:10 ↔ 0.25x20 Washer:19
- Insert:66: 90630A110:9 ↔ 0.25x20 Washer:20
- Insert:67: 90630A110:12 ↔ 0.25x20 Washer:27
- Insert:68: 90630A110:11 ↔ 0.25x20 Washer:28
- Insert:69: 90630A110:13 ↔ 0.25x20 Washer:30
- Insert:70: 90630A110:14 ↔ 0.25x20 Washer:29
- Insert:71: 90630A110:15 ↔ 0.25x20 Washer:32
- Insert:72: 90630A110:16 ↔ 0.25x20 Washer:31
- Insert:73: 90630A110:17 ↔ 0.25x20 Washer:36
- Insert:74: 90630A110:18 ↔ 0.25x20 Washer:35
- Insert:75: 90630A110:19 ↔ 0.25x20 Washer:34
- Insert:76: 90630A110:20 ↔ 0.25x20 Washer:33